# Autodesk Inventor assembly: левый привод_MIR
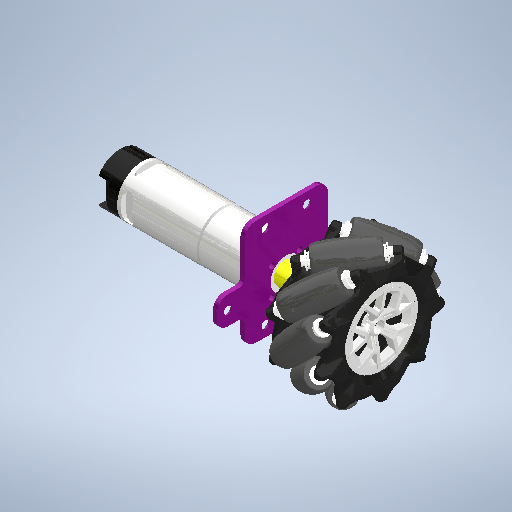
[picture p0: Inventor's stored thumbnail of the model, 512x512]
Saved by Autodesk Inventor 2025 (Build 290162000, 162)
## iProperties
Created: 2025-02-16
Part Number: левый привод_MIR
Document SubType Name: Assembly
Designer: volko
Author: volko
## Documents named in this file (5)
- C:\Users\volko\Desktop\диплом\Модели\детали\левый привод_MIR.iam
- C:\Users\volko\Desktop\диплом\Модели\детали\CHP-42GP-775 ABHL_MIR_MIR.ipt
- C:\Users\volko\Desktop\диплом\Модели\детали\переходная втулка_MIR_MIR.ipt
- C:\Users\volko\Desktop\диплом\Модели\Mecanum wheel - left\Mecanum wheel - left_MIR.iam
- C:\Users\volko\Desktop\диплом\Модели\детали\кронштейн_zerkalo.ipt
## Components (4 placed, 4 different names)
1. CHP-42GP-775 ABHL_MIR_MIR:1 — Заподлицо:1, Совмещение:2, Совмещение:1, Совмещение:4, Совмещение:3, Совмещение:12
2. переходная втулка_MIR_MIR:1 — Совмещение:4, Совмещение:3, Совмещение:10, Совмещение:9, Совмещение:8, Совмещение:11
3. Mecanum wheel - left_MIR:1 [sub-assembly] — Совмещение:10, Совмещение:9, Совмещение:8
4. кронштейн_zerkalo:1 — Совмещение:11, Совмещение:12
## Relationships (10: Mate 9, Flush 1)
- Заподлицо:1 [Flush]: CHP-42GP-775 ABHL_MIR_MIR:1
- Совмещение:2 [Mate]: CHP-42GP-775 ABHL_MIR_MIR:1
- Совмещение:1 [Mate]: CHP-42GP-775 ABHL_MIR_MIR:1
- Совмещение:4 [Mate]: CHP-42GP-775 ABHL_MIR_MIR:1 ↔ переходная втулка_MIR_MIR:1
- Совмещение:3 [Mate]: CHP-42GP-775 ABHL_MIR_MIR:1 ↔ переходная втулка_MIR_MIR:1
- Совмещение:10 [Mate]: переходная втулка_MIR_MIR:1 ↔ Mecanum wheel - left_MIR:1
- Совмещение:9 [Mate]: переходная втулка_MIR_MIR:1 ↔ Mecanum wheel - left_MIR:1
- Совмещение:8 [Mate]: переходная втулка_MIR_MIR:1 ↔ Mecanum wheel - left_MIR:1
- Совмещение:11 [Mate]: переходная втулка_MIR_MIR:1 ↔ кронштейн_zerkalo:1
- Совмещение:12 [Mate]: CHP-42GP-775 ABHL_MIR_MIR:1 ↔ кронштейн_zerkalo:1
